# Autodesk Inventor assembly: GEABA1.0-80-10-B-10-KFC30-K3
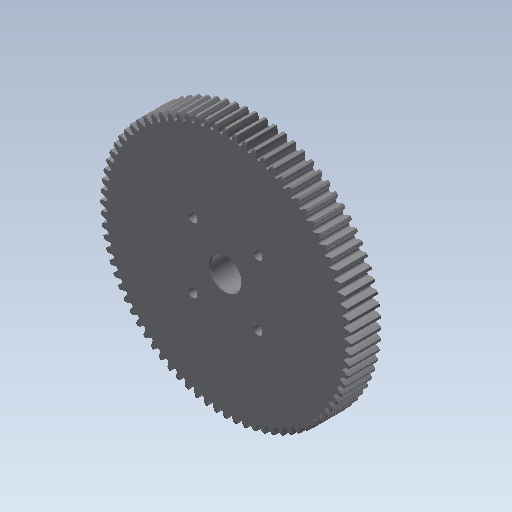
[picture p0: Inventor's stored thumbnail of the model, 512x512]
Saved by Autodesk Inventor 2020.2 (Build 242310000, 310)
## iProperties
Created: 2022-11-02
Part Number: GEABA1.0-80-10-B-10-KFC30-K3
Catalog Web Link: www.cadenas.de
Description: GEABM, GEABMS, GEABMT, GEABP, GEABPS, GEABPT, GEABA, GEABAS, GEABAT-Plastic Spur Gears - Pressure Angle 20 Degrees, Module 0.5/0.8/1.0/1.5/2.0/2.5/3.0
Vendor: MISUMI
Document SubType Name: Assembly
Designer: psAdmin
Manufacturer: MISUMI
Mass: 60.3551 g
Surface Area: 175.026 cm^2
Volume: 60.3551 cm^3
Density: 1 g/cm^3
Category: PARTsolutions
Company: MISUMI
PSOL_IDENT_0: {$CADENAS_DATA/23d-libs/misumi/metric/54_spur_gears/geabms20_asmtab.prj},415 {VTYP=3D},{STYP=ASSTAB}
PSOL_IDENT_1: ,{NB=GEABA1.0-80-10-B-10-KFC30-K3},{LINA=GEABA1.0-80-10-B-10-KFC30-K3},{NN=GEABM, GEABMS, GEABMT, GE
PSOL_IDENT_2: ABP, GEABPS, GEABPT, GEABA, GEABAS, GEABAT},{DATE=16.08.2021 10:08:31},{GEOMDATE=16.08.2021 10:08:28
PSOL_IDENT_3: },{VERSION=},{LINEID=30},{WBVAR=MATSG,MATCR,NT,B,TS,PS,ALT1,ALT2,TPC,ALT11,ALT10,BS,ALT3,Z,J,ALT4,Q,
PSOL_IDENT_4: R,S,T,ALT5,LFC,LTC,MALT5,ALT6,KFC,KTC,K},{WBNUMERIC=NT,B,BS,Z,J,Q,R,S,T,LFC,LTC,KFC,KTC,K}  {NB=GEAB
PSOL_IDENT_5: A1.0-80-10-B-10-KFC30-K3},{LINA=GEABA1.0-80-10-B-10-KFC30-K3},{KT=DUMMY},{PN=GEABA1.0-80-10-B-10-KFC
PSOL_IDENT_6: 30-K3},{TYPE=GEABA},{MATSG=PB},{MATSGALG='MCN','MC Nylon','PW','Polyacetal White','PB','Polyacetal B
PSOL_IDENT_7: lue'},{MATCR=},{MATCRALG='','-','S45C','1045 Carbon Steel','SUS304','304 Stainless Steel'},{MOD=1.0}
PSOL_IDENT_8: ,{MOD1=1.0},{NT=80},{NTALG=15,16,18,20,22,24,25,26,28,30,32,35,36,40,45,48,50,55,60,70,75,80,90,100,
PSOL_IDENT_9: 120},{B=10},{BALG=10,15},{TS=B},{TSALG='A','A','B','B'},{TSPN=-B},{PS=10},{PSALG='10','10','11','11'
PSOL_IDENT_10: ,'12','12','13','13','14','14','15','15','16','16','17','17','18','18','19','19','20','20','21','21'
PSOL_IDENT_11: ,'22','22','23','23','24','24','25','25','26','26','27','27','28','28'},{PSCRL='10','10','11','11','
PSOL_IDENT_12: 12','12','13','13','14','14','15','15','16','16','17','17','18','18','19','19','20','20','21','21','
PSOL_IDENT_13: 22','22','23','23','24','24','25','25','26','26','27','27','28','28'},{PSCRW='10','10','12','12','15'
PSOL_IDENT_14: ,'15','20','20'},{DD=80.0},{DD05=40},{DD08=64},{DD10=80},{DD15=120},{DD20=0},{DD25=0},{DD30=0},{D=82
PSOL_IDENT_15: .0},{D05=41},{D08=65.6},{D10=82},{D15=123},{D20=0},{D25=0},{D30=0},{G=77.50},{G05=38.75},{G08=62},{G
PSOL_IDENT_16: 10=77.5},{G15=116.25},{G20=0},{G25=0},{G30=0},{H=40.0},{L=20},{LL1=10},{LL2=4.0},{M=M4},{M3D=4},{P=1
PSOL_IDENT_17: 0.00},{DD1=0},{CIFR=15},{CIFM=4},{CIFK=0},{CIFTAP=1},{SCREW=4.000},{SCREWL=3.000},{ALT1=},{ALT1ALG=''
PSOL_IDENT_18: ,'w/o Set Screw','KC90','with KC90 (Set Screw)','KC120','with KC120 (Set Screw)'},{ALT1PN=},{ALT2=},
PSOL_IDENT_19: {ALT2ALG='','w/o TPC (Tapped Hole Dimension)','TPC','with TPC (Tapped Hole Dimension)'},{TPC=N/A},{T
PSOL_IDENT_20: PCALG='N/A'},{ALT2PN=},{KC=0},{ALT11=},{ALT11ALG='', 'w/o GBA (Gear bottom adjustment of phase focus
PSOL_IDENT_21: )', 'GBA', 'with GBA (Gear bottom adjustment of phase focus)' },{ALT11PN=},{DEG=0},{ALT10=},{ALT10AL
PSOL_IDENT_22: G= '','w/o BS (Boss Cut)','BS','with BS (Boss Cut)' },{ALT10PN=},{BS=0.0},{BSALG=0},{BSMIN=7.000},{B
PSOL_IDENT_23: SMINALG=7},{BSMAX=10},{LL13D=10},{LL23D=16},{ALT3=},{ALT3ALG= '','w/o Stepped Hole','DHL','with DHL
PSOL_IDENT_24: (Stepped Hole)','DHR','with DHR (Stepped Hole)' },{ALT3PN=},{ZJPN=},{ALT31=1},{ALT32=1},{Z=0},{ZALG=
PSOL_IDENT_25: 0},{ZMINL=12},{ZMAXL=73},{ZMINR=12},{ZMAXR=36},{ZPN=},{J=0.0},{JALG=0},{JMIN=2},{JMAX=0},{JPN=},{ALT
PSOL_IDENT_26: 4=},{ALT4ALG= '','w/o WDH (Both Ends Stepped Hole)','WDH','with WDH (Both Ends Stepped Hole)' },{ALT
PSOL_IDENT_27: 4PN=},{QRSTPN=},{LB=20.000},{Q=0},{QALG=0},{QMIN=12},{QMAX=36},{QPN=},{R=0},{RALG=0},{RMIN=12},{RMAX=
PSOL_IDENT_28: 36},{RPN=},{S=0},{SALG=0},{SMIN=3},{SMAX=14},{SPN=},{T=0},{TALG=0},{TMIN=3},{TMAX=0},{TPN=},{ALT5=},
PSOL_IDENT_29: {ALT5ALG= '','Not applicable' },{LFC=0},{LFCALG=0},{LTC=0},{LTCALG=0},{LPCDMIN=18},{LPCDMAX=70},{LCM
PSOL_IDENT_30: AX=73},{MALT5=N/A},{MALT5ALG= 'N/A' },{LCMAX2=70},{C=0.0},{ALT5PN=},{ALT6=KFC},{ALT6ALG= '','w/o Sid
PSOL_IDENT_31: e Through Hole','KFC','with KFC (Side Through Hole)','KTC','with KTC (Side Through Hole)' },{ALT6PN=
PSOL_IDENT_32: -KFC},{KFTCPN=30-K3},{KFC=30},{KFCALG=[17:33/1],[47:70/1]},{KFCPN=30},{KTC=0},{KTCALG=[0]},{KTCPN=},
PSOL_IDENT_33: {KPCDMIN1=17},{KPCDMAX1=33},{KPCDMIN2=47},{KPCDMAX2=70},{K=3.0},{KALG=[3:6/0.5]},{KPCD=30},{KPN=-K3}
PSOL_IDENT_34: ,{AG=0},{LBS=20},{PCD=30},{SHN=4},{SHDEG1=45},{SHDEG2=90},{PZQRDD2=10},{PPATH=geabms20/geabms20_asmt
PSOL_IDENT_35: pl.prj}
NB: GEABA1.0-80-10-B-10-KFC30-K3
NN: GEABM, GEABMS, GEABMT, GEABP, GEABPS, GEABPT, GEABA, GEABAS, GEABAT
NT: 80
NBSYN: $PN.
LINA: GEABA1.0-80-10-B-10-KFC30-K3
CATALOG: Misumi
PN: GEABA1.0-80-10-B-10-KFC30-K3
MATSG: Polyacetal Blue
MATCR: -
MOD: 1.0
B: 10
TS: B
PS: 10
DD: 80
D: 82
G: 77.5
H: 40
L: 20
LL1: 10
LL2: 4
M: M4
DD1: 0
ALT1: w/o Set Screw
ALT2: w/o TPC (Tapped Hole Dimension)
TPC: N/A
ALT11: w/o GBA (Gear bottom adjustment of phase focus)
ALT10: w/o BS (Boss Cut)
BS: 0
ALT3: w/o Stepped Hole
Z: 0
J: 0
ALT4: w/o WDH (Both Ends Stepped Hole)
Q: 0
R: 0
S: 0
T: 0
ALT5: Not applicable
LFC: 0
LTC: 0
MALT5: N/A
C: 0
ALT6: with KFC (Side Through Hole)
KFC: 30
KTC: 0
K: 3
SUPPLIER: MISUMI
ARTICLENO: GEABA1.0-80-10-B-10-KFC30-K3
BOMINFO: GEABA1.0-80-10-B-10-KFC30-K3
CREATOR: CADENAS GmbH
Title: GEABA1.0-80-10-B-10-KFC30-K3
Author: Cadenas PARTsolutions
Comments: Plastic Spur Gears - Pressure Angle 20 Degrees, Module 0.5/0.8/1.0/1.5/2.0/2.5/3.0
## Documents named in this file (3)
- C:\Users\Administrator\Documents\kamuy2\Parts\GEABA1.0-80-10-B-10-KFC30-K3_Autodesk_Inventor_2020_20221102\AIS2020\GEABA1_0-80-10-B-10-KFC30-K3.iam
- C:\Users\Administrator\Documents\kamuy2\Parts\GEABA1.0-80-10-B-10-KFC30-K3_Autodesk_Inventor_2020_20221102\AIS2020\GEABA1_0-80-10-B-10-KFC30-K3_b.ipt
- C:\Users\Administrator\Documents\kamuy2\Parts\GEABA1.0-80-10-B-10-KFC30-K3_Autodesk_Inventor_2020_20221102\AIS2020\SET-SCREW4-3.ipt
## Components (2 placed, 2 different names)
1. GEABA1_0-80-10-B-10-KFC30-K3_b:1 — gear_to_screw_XY@1 <-> CP_XY@2, gear_to_screw_Z@1 <-> CP_Z@2, gear_to_screw_YZ@1 <-> CP_YZ@2
2. SET-SCREW4-3:1 — gear_to_screw_XY@1 <-> CP_XY@2, gear_to_screw_Z@1 <-> CP_Z@2, gear_to_screw_YZ@1 <-> CP_YZ@2
## Relationships (3: Mate 2, Angle 1)
- gear_to_screw_XY@1 <-> CP_XY@2 [Mate]: GEABA1_0-80-10-B-10-KFC30-K3_b:1 ↔ SET-SCREW4-3:1
- gear_to_screw_Z@1 <-> CP_Z@2 [Mate]: GEABA1_0-80-10-B-10-KFC30-K3_b:1 ↔ SET-SCREW4-3:1
- gear_to_screw_YZ@1 <-> CP_YZ@2 [Angle] (0 deg): GEABA1_0-80-10-B-10-KFC30-K3_b:1 ↔ SET-SCREW4-3:1
